# Autodesk Inventor assembly: 90 Barcket
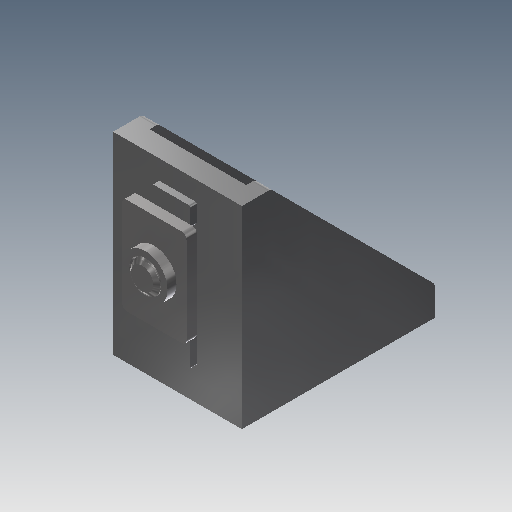
[picture p0: Inventor's stored thumbnail of the model, 512x512]
Saved by Autodesk Inventor 2017 (Build 210142000, 142)
## iProperties
Created: 2015-06-02
Part Number: 90 Barcket
Document SubType Name: Assembly
Designer: Sawaiz Syed
Author: Sawaiz Syed
## Documents named in this file (4)
- C:\Users\sawaiz\oneDrive\projects\muonTelescope\frame\brackets\angleBracket.iam
- C:\Users\sawaiz\oneDrive\projects\muonTelescope\frame\brackets\angleBracket.ipt
- C:\Users\sawaiz\oneDrive\projects\muonTelescope\frame\brackets\m5x10.ipt
- C:\Users\sawaiz\oneDrive\projects\muonTelescope\frame\brackets\m5TNut.ipt
## Components (5 placed, 3 different names)
1. angleBracket:1 — Mate:11, Angle:3, Mate:12, Mate:13, Mate:14, Mate:15, Angle:4, Mate:19
2. m5x10:1 — Mate:12, Mate:14, Mate:18
3. m5x10:2 — Mate:13, Mate:15, Mate:17
4. m5TNut:2 — Mate:11, Angle:3, Mate:17
5. m5TNut:3 — Mate:18, Angle:4, Mate:19
## Relationships (10: Mate 8, Angle 2)
- Mate:11 (2 mm): angleBracket:1 ↔ m5TNut:2
- Angle:3 (0 deg): angleBracket:1 ↔ m5TNut:2
- Mate:12: angleBracket:1 ↔ m5x10:1
- Mate:13: angleBracket:1 ↔ m5x10:2
- Mate:14: angleBracket:1 ↔ m5x10:1
- Mate:15: angleBracket:1 ↔ m5x10:2
- Mate:17: m5x10:2 ↔ m5TNut:2
- Mate:18: m5x10:1 ↔ m5TNut:3
- Angle:4 (0 deg): angleBracket:1 ↔ m5TNut:3
- Mate:19 (2 mm): angleBracket:1 ↔ m5TNut:3
